# Autodesk Inventor assembly: schreibtisch
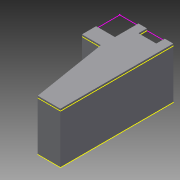
[picture p0: Inventor's stored thumbnail of the model, 180x180]
Saved by Autodesk Inventor 2013 (Build 170138000, 138)
## iProperties
Created: 2014-03-27
Part Number: schreibtisch
Document SubType Name: Assembly
Designer: hhanff
Author: hhanff
## Documents named in this file (8)
- C:\Users\hhanff\Dropbox\src\inventor\schreibtisch\schreibtisch.iam
- C:\Users\hhanff\Dropbox\src\inventor\schreibtisch\rueckteil.ipt
- C:\Users\hhanff\Dropbox\src\inventor\schreibtisch\schreibtischplatte.ipt
- C:\Users\hhanff\Dropbox\src\inventor\schreibtisch\regalboden.ipt
- C:\Users\hhanff\Dropbox\src\inventor\schreibtisch\schreibtischplatte top.ipt
- C:\Users\hhanff\Dropbox\src\inventor\schreibtisch\seitenteil_rechts.ipt
- C:\Users\hhanff\Dropbox\src\inventor\schreibtisch\seitenteil_links.ipt
- C:\Users\hhanff\Dropbox\src\inventor\schreibtisch\deckel.ipt
## Components (9 placed, 7 different names)
1. seitenteil_links:1 — Mate:26, Mate:27, Mate:28, Mate:33, Mate:34, Mate:35, Mate:36
2. seitenteil_rechts:1 — Mate:23, Mate:24, Mate:25, Mate:29, Mate:31, Mate:38, Mate:40, Mate:41
3. rueckteil:1 — Mate:23, Mate:24, Mate:25, Mate:26, Mate:27, Mate:30, Mate:32, Mate:37, Mate:39, Mate:42
4. schreibtischplatte:2 — Mate:34, Mate:35, Mate:36
5. regalboden:1 — Mate:41, Mate:42
6. regalboden:2 — Mate:37, Mate:38
7. regalboden:3 — Mate:39, Mate:40
8. schreibtischplatte top:1 — Mate:28, Mate:29, Mate:30
9. deckel:1 — Mate:31, Mate:32, Mate:33
## Relationships (20: Mate 20)
- Mate:23: seitenteil_rechts:1 ↔ rueckteil:1
- Mate:24: seitenteil_rechts:1 ↔ rueckteil:1
- Mate:25: seitenteil_rechts:1 ↔ rueckteil:1
- Mate:26: seitenteil_links:1 ↔ rueckteil:1
- Mate:27: seitenteil_links:1 ↔ rueckteil:1
- Mate:28: seitenteil_links:1 ↔ schreibtischplatte top:1
- Mate:29: seitenteil_rechts:1 ↔ schreibtischplatte top:1
- Mate:30: rueckteil:1 ↔ schreibtischplatte top:1
- Mate:31: seitenteil_rechts:1 ↔ deckel:1
- Mate:32: rueckteil:1 ↔ deckel:1
- Mate:33: seitenteil_links:1 ↔ deckel:1
- Mate:34: seitenteil_links:1 ↔ schreibtischplatte:2
- Mate:35: seitenteil_links:1 ↔ schreibtischplatte:2
- Mate:36: seitenteil_links:1 ↔ schreibtischplatte:2
- Mate:37: rueckteil:1 ↔ regalboden:2
- Mate:38: seitenteil_rechts:1 ↔ regalboden:2
- Mate:39: rueckteil:1 ↔ regalboden:3
- Mate:40: seitenteil_rechts:1 ↔ regalboden:3
- Mate:41: seitenteil_rechts:1 ↔ regalboden:1
- Mate:42: rueckteil:1 ↔ regalboden:1
